# Autodesk Inventor assembly: Car
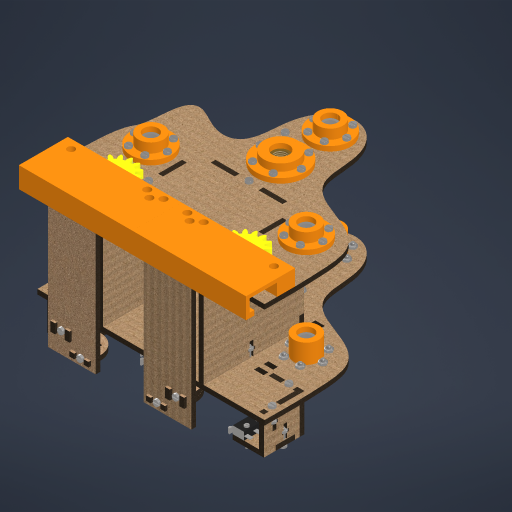
[picture p0: Inventor's stored thumbnail of the model, 512x512]
Saved by Autodesk Inventor 2024.1 (Build 281209000, 209)
## iProperties
Created: 2023-08-04
Part Number: Car
Document SubType Name: Assembly
Designer: jaege
Author: jaege
## Documents named in this file (35)
- C:\Users\jaege\VUB\Schakel_Ind_Elo\Year_1_Both\BA_Thesis\3D_Files\Lift_V2\Car_ASM.iam
- C:\Users\jaege\VUB\Schakel_Ind_Elo\Year_1_Both\BA_Thesis\3D_Files\Lift_V2\Cart_Floor.ipt
- C:\Users\jaege\VUB\Schakel_Ind_Elo\Year_1_Both\BA_Thesis\3D_Files\Lift_V2\Spindle_Block_ASM.iam
- C:\Users\jaege\VUB\Schakel_Ind_Elo\Year_1_Both\BA_Thesis\3D_Files\Lift_V2\Servo_Motor.ipt
- C:\Users\jaege\VUB\Schakel_Ind_Elo\Year_1_Both\BA_Thesis\3D_Files\Lift_V2\Bearing_ASM.iam
- C:\Users\jaege\VUB\Schakel_Ind_Elo\Year_1_Both\BA_Thesis\3D_Files\Lift_V2\Door.ipt
- C:\Users\jaege\VUB\Schakel_Ind_Elo\Year_1_Both\BA_Thesis\3D_Files\Lift_V2\Gear.ipt
- C:\Users\jaege\VUB\Schakel_Ind_Elo\Year_1_Both\BA_Thesis\3D_Files\Lift_V2\Lever.ipt
- C:\Users\jaege\VUB\Schakel_Ind_Elo\Year_1_Both\BA_Thesis\3D_Files\Lift_V2\Receptacle.ipt
- C:\Users\jaege\VUB\Schakel_Ind_Elo\Year_1_Both\BA_Thesis\3D_Files\Lift_V2\Shaft.ipt
- C:\Users\jaege\Documents\Inventor\Content Center Files\R2024\en-US\ISO 1207(2)\ISO 1207 - M3 x 12.ipt
- C:\Users\jaege\Documents\Inventor\Content Center Files\R2024\en-US\ISO 4032(2)\ISO 4032 - M3 - ISO.ipt
- C:\Users\jaege\Documents\Inventor\Content Center Files\R2024\en-US\ISO 7089\ISO 7089 - 3 - 140 HV(1).ipt
- C:\Users\jaege\Documents\Inventor\Content Center Files\R2024\en-US\ISO 1207(2)\ISO 1207 - M3 x 8.ipt
- C:\Users\jaege\VUB\Schakel_Ind_Elo\Year_1_Both\BA_Thesis\3D_Files\Lift_V2\Shaft_MIR.ipt
- C:\Users\jaege\VUB\Schakel_Ind_Elo\Year_1_Both\BA_Thesis\3D_Files\Lift_V2\Receptacle_MIR.ipt
- C:\Users\jaege\VUB\Schakel_Ind_Elo\Year_1_Both\BA_Thesis\3D_Files\Lift_V2\Door_MIR.ipt
- C:\Users\jaege\VUB\Schakel_Ind_Elo\Year_1_Both\BA_Thesis\3D_Files\Lift_V2\Car_Left.ipt
- C:\Users\jaege\VUB\Schakel_Ind_Elo\Year_1_Both\BA_Thesis\3D_Files\Lift_V2\Car_Rear.ipt
- C:\Users\jaege\VUB\Schakel_Ind_Elo\Year_1_Both\BA_Thesis\3D_Files\Lift_V2\Cart_Floor_Bottom.ipt
- C:\Users\jaege\VUB\Schakel_Ind_Elo\Year_1_Both\BA_Thesis\3D_Files\Lift_V2\Spindle_Block_ASM_MIR.iam
- C:\Users\jaege\VUB\Schakel_Ind_Elo\Year_1_Both\BA_Thesis\3D_Files\Lift_V2\Bearing_ASM_MIR1.iam
- C:\Users\jaege\VUB\Schakel_Ind_Elo\Year_1_Both\BA_Thesis\3D_Files\Lift_V2\Magnet_Holder.ipt
- C:\Users\jaege\VUB\Schakel_Ind_Elo\Year_1_Both\BA_Thesis\3D_Files\Lift_V2\LimitSwitch_Small.ipt
- C:\Users\jaege\VUB\Schakel_Ind_Elo\Year_1_Both\BA_Thesis\3D_Files\Lift_V2\Door_LimitSwitch_Offset.ipt
- C:\Users\jaege\VUB\Schakel_Ind_Elo\Year_1_Both\BA_Thesis\3D_Files\Lift_V2\Door_LimitSwitch_Holder_Side_1.ipt
- C:\Users\jaege\VUB\Schakel_Ind_Elo\Year_1_Both\BA_Thesis\3D_Files\Lift_V2\Door_LimitSwitch_Holder_Side_2.ipt
- C:\Users\jaege\VUB\Schakel_Ind_Elo\Year_1_Both\BA_Thesis\3D_Files\Lift_V2\Door_LimitSwitch_Holder_Plate.ipt
- C:\Users\jaege\VUB\Schakel_Ind_Elo\Year_1_Both\BA_Thesis\3D_Files\Lift_V2\Door_LimitSwitch_Holder_Side_1_MIR.ipt
- C:\Users\jaege\VUB\Schakel_Ind_Elo\Year_1_Both\BA_Thesis\3D_Files\Lift_V2\Door_LimitSwitch_Holder_Side_2_MIR.ipt
- C:\Users\jaege\VUB\Schakel_Ind_Elo\Year_1_Both\BA_Thesis\3D_Files\Lift_V2\Door_LimitSwitch_Holder_Plate_MIR.ipt
- C:\Users\jaege\Documents\Inventor\Content Center Files\R2024\en-US\AS 1427(10)\AS 1427 - M2 x 25(7).ipt
- C:\Users\jaege\Documents\Inventor\Content Center Files\R2024\en-US\ISO 7089\ISO 7089 - 2 - 140 HV(1).ipt
- C:\Users\jaege\Documents\Inventor\Content Center Files\R2024\en-US\ISO 4032(2)\ISO 4032 - M2 - ISO.ipt
- C:\Users\jaege\Documents\Inventor\Content Center Files\R2024\en-US\AS 1427(10)\AS 1427 - M2 x 16(7).ipt
## Components (234 placed, 35 different names)
1. Spindle_Block_ASM:1 [sub-assembly]
2. Servo_Motor:1 — Mate:433, Mate:434, Mate:435
3. Bearing_ASM:1 [sub-assembly]
4. Bearing_ASM:2 [sub-assembly]
5. Door:1 — Mate:245, Mate:246, Mate:295, Mate:296, Mate:297, Mate:312, Mate:313, Mate:314, Mate:316, Mate:317, Mate:318
6. Gear:1
7. Lever:1 — Mate:245
8. Lever:2 — Mate:246, Mate:311, Mate:319
9. Receptacle:1 — Angle:20
10. Shaft:1
11. Bearing_ASM:3 [sub-assembly]
12. Servo_Motor:2 — Mate:436, Mate:437
13. Gear:2
14. Shaft_MIR:1
15. Receptacle_MIR:1 — Angle:21, Angle:23, Mate:438, Mate:439, Mate:440, Mate:441, Mate:442, Mate:443, Mate:444, Mate:446, Mate:448, Mate:450, Mate:451, Mate:452, Mate:453, Mate:454
16. Door_MIR:1 — Mate:299, Mate:300, Mate:320, Mate:321, Mate:322, Mate:324, Mate:325, Mate:326
17. Lever:3 — Mate:294, Mate:301, Mate:323
18. Lever:4 — Mate:298
19. Cart_Floor:1 — Flush:6, Mate:166, Mate:167, Mate:168, Mate:169, Flush:8, Symmetry:1, Mate:261, Mate:263, Mate:278, Mate:393, Mate:394, Mate:395, Mate:405, Mate:406, Mate:407, Mate:408, Mate:409, Mate:410, Mate:411, Mate:413, Mate:415, Mate:429, Mate:430, Mate:431, Mate:432, Mate:445, Mate:447, Mate:449, Mate:450, Mate:451, Mate:455
20. Car_Left:1 — Flush:6, Flush:7, Mate:262, Mate:263, Mate:264, Symmetry:2, Mate:412, Mate:414, Mate:416, Angle:13, Angle:15
21. Car_Right:2 — Mate:166, Mate:167, Mate:168, Mate:169, Symmetry:2, Mate:402, Mate:404, Angle:12, Angle:14, Angle:16
22. Car_Rear:1 — Flush:7, Mate:170, Mate:171, Mate:261, Mate:262, Mate:397, Mate:398, Mate:399, Mate:400, Mate:401, Mate:403, Mate:424, Mate:426, Mate:428, Angle:17, Angle:18
23. Cart_Floor_Bottom:1 — Mate:170, Mate:171, Flush:8, Symmetry:1, Mate:244, Flush:9, Mate:247, Mate:264, Mate:265, Mate:266, Mate:267, Mate:268, Mate:269, Mate:270, Mate:271, Mate:272, Mate:273, Mate:274, Mate:275, Mate:276, Mate:277, Mate:279, Mate:280, Mate:281, Mate:282, Mate:283, Mate:284, Flush:35, Mate:285, Mate:286, Mate:287, Flush:36, Mate:288, Mate:305, Mate:307, Mate:331, Mate:335, Mate:339, Mate:343, Mate:360, Mate:361, Mate:362, Mate:364, Mate:365, Mate:366, Mate:376, Mate:377, Mate:378, Mate:380, Mate:381, Mate:382, Mate:383, Mate:417, Mate:418, Mate:419, Mate:420, Mate:421, Mate:422, Mate:423, Mate:425, Mate:427
24. Spindle_Block_ASM_MIR:1 [sub-assembly] — Mate:181, Mate:182, Mate:183, Mate:184, Mate:185, Mate:186, Mate:187, Mate:188, Mate:189, Mate:208, Mate:209, Mate:210, Mate:211, Mate:212, Mate:213, Mate:214, Mate:215, Mate:216, Mate:265, Mate:266
25. Bearing_ASM_MIR1:1 [sub-assembly] — Mate:190, Mate:191, Mate:192, Mate:193, Mate:194, Mate:195, Mate:196, Mate:197, Mate:198, Mate:199, Mate:200, Mate:201, Mate:202, Mate:203, Mate:204, Mate:205, Mate:206, Mate:207, Mate:271, Mate:274
26. Bearing_ASM_MIR1:2 [sub-assembly] — Mate:172, Mate:173, Mate:174, Mate:175, Mate:176, Mate:177, Mate:178, Mate:179, Mate:180, Mate:217, Mate:218, Mate:219, Mate:220, Mate:221, Mate:222, Mate:223, Mate:224, Mate:225, Mate:267, Mate:268
27. Bearing_ASM_MIR1:3 [sub-assembly] — Mate:226, Mate:227, Mate:228, Mate:229, Mate:230, Mate:231, Mate:232, Mate:233, Mate:234, Mate:235, Mate:236, Mate:237, Mate:238, Mate:239, Mate:240, Mate:241, Mate:242, Mate:243, Mate:272, Mate:273
28. LimitSwitch_Small:1 — Mate:250, Mate:251, Mate:252, Mate:258, Mate:259, Mate:260
29. LimitSwitch_Small:6 — Mate:308, Mate:309, Mate:310, Mate:311, Mate:344, Mate:345, Mate:346, Mate:348, Mate:349, Mate:350
30. LimitSwitch_Small:3 — Mate:258, Mate:259, Mate:260, Mate:281, Mate:282, Mate:328, Mate:329, Mate:330, Mate:332, Mate:333, Mate:334
31. LimitSwitch_Small:4 — Mate:255, Mate:256, Mate:257, Mate:283, Mate:284, Mate:336, Mate:337, Mate:338, Mate:340, Mate:341, Mate:342
32. LimitSwitch_Small:5 — Mate:290, Mate:291, Mate:292, Mate:294, Mate:301, Mate:352, Mate:353, Mate:354, Mate:356, Mate:357, Mate:358
33. LimitSwitch_Small:2 — Mate:249, Mate:253, Mate:254, Mate:255, Mate:256, Mate:257
34. Magnet_Holder:1 — Mate:244, Mate:278, Mate:279, Mate:280, Mate:396, Angle:19
35. Door_LimitSwitch_Offset:1 — Flush:9, Mate:248, Flush:10, Mate:249, Mate:253, Mate:254
36. Door_LimitSwitch_Offset:2 — Mate:247, Mate:248, Flush:10, Mate:250, Mate:251, Mate:252
37. Door_LimitSwitch_Holder_Side_1:1 — Flush:35, Mate:285, Mate:286, Mate:287, Mate:289, Flush:37, Flush:38, Flush:39, Mate:367, Mate:371, Angle:10
38. Door_LimitSwitch_Holder_Side_2:1 — Flush:36, Mate:288, Mate:289, Flush:37, Mate:293, Flush:40, Mate:363, Mate:375, Angle:8
39. Door_LimitSwitch_Holder_Plate:1 — Flush:38, Mate:290, Mate:291, Mate:292, Mate:293, Flush:39, Flush:40, Mate:355, Mate:359, Mate:368, Mate:369, Mate:370, Mate:372, Mate:373, Mate:374
40. Lever:5 — Mate:295, Mate:296, Mate:297, Mate:315, Angle:6
41. Lever:6 — Mate:298, Mate:299, Mate:300, Mate:327
42. Door_LimitSwitch_Holder_Side_1_MIR:1 — Flush:41, Mate:302, Flush:43, Mate:304, Mate:305, Flush:44, Mate:307, Mate:380, Mate:384, Mate:388, Angle:2
43. Door_LimitSwitch_Holder_Side_2_MIR:1 — Flush:41, Mate:302, Flush:42, Mate:303, Flush:44, Mate:379, Mate:392, Angle:3
44. Door_LimitSwitch_Holder_Plate_MIR:1 — Flush:42, Flush:43, Mate:303, Mate:304, Mate:308, Mate:309, Mate:310, Mate:347, Mate:351, Mate:385, Mate:386, Mate:387, Mate:389, Mate:390, Mate:391
45. ISO 1207 M3 x 12:53 — Mate:312, Mate:313
46. ISO 4032 M3:53 — Mate:314, Mate:315, Angle:5, Angle:6, Angle:11
47. ISO 1207 M3 x 12:54 — Mate:316, Mate:317
48. ISO 4032 M3:54 — Mate:318, Mate:319, Angle:5, Angle:11
49. ISO 1207 M3 x 12:55 — Mate:320, Mate:321
50. ISO 4032 M3:55 — Mate:322, Mate:323
51. ISO 1207 M3 x 12:56 — Mate:324, Mate:325
52. ISO 4032 M3:56 — Mate:326, Mate:327
53. AS 1427 (8) - Metric M2 x 25:1 — Mate:328, Mate:329
54. ISO 7089 2:1 — Mate:330, Mate:331, Insert:5
55. ISO 4032 M2:1 — Insert:5
56. AS 1427 (8) - Metric M2 x 25:2 — Mate:332, Mate:333
57. ISO 7089 2:2 — Mate:334, Mate:335, Insert:6
58. ISO 4032 M2:2 — Insert:6
59. AS 1427 (8) - Metric M2 x 25:3 — Mate:336, Mate:337
60. ISO 7089 2:3 — Mate:338, Mate:339, Insert:7
61. ISO 4032 M2:3 — Insert:7
62. AS 1427 (8) - Metric M2 x 25:4 — Mate:340, Mate:341
63. ISO 7089 2:4 — Mate:342, Mate:343, Insert:8
64. ISO 4032 M2:4 — Insert:8
65. AS 1427 (8) - Metric M2 x 16:1 — Mate:344, Mate:345
66. ISO 7089 2:5 — Mate:346, Mate:347, Insert:9
67. ISO 4032 M2:5 — Insert:9
68. AS 1427 (8) - Metric M2 x 16:2 — Mate:348, Mate:349
69. ISO 7089 2:6 — Mate:350, Mate:351, Insert:10
70. ISO 4032 M2:6 — Insert:10
71. AS 1427 (8) - Metric M2 x 16:3 — Mate:352, Mate:353
72. ISO 7089 2:7 — Mate:354, Mate:355, Insert:11
73. ISO 4032 M2:7 — Insert:11
74. AS 1427 (8) - Metric M2 x 16:4 — Mate:356, Mate:357
75. ISO 7089 2:8 — Mate:358, Mate:359, Insert:12
76. ISO 4032 M2:8 — Insert:12
77. ISO 1207 M3 x 12:57 — Mate:360, Mate:361
78. ISO 4032 M3:57 — Mate:362, Mate:363, Angle:7, Angle:8
79. ISO 1207 M3 x 12:58 — Mate:364, Mate:365
80. ISO 4032 M3:58 — Mate:366, Mate:367, Angle:9, Angle:10
81. ISO 1207 M3 x 12:59 — Mate:368, Mate:369
82. ISO 4032 M3:59 — Mate:370, Mate:371, Angle:9
83. ISO 1207 M3 x 12:60 — Mate:372, Mate:373
84. ISO 4032 M3:60 — Mate:374, Mate:375, Angle:7
85. ISO 1207 M3 x 12:61 — Mate:376, Mate:377
86. ISO 4032 M3:61 — Mate:378, Mate:379, Angle:4
87. ISO 1207 M3 x 12:62 — Mate:381, Mate:382
88. ISO 4032 M3:62 — Mate:383, Mate:384, Angle:1
89. ISO 1207 M3 x 12:63 — Mate:385, Mate:386
90. ISO 4032 M3:63 — Mate:387, Mate:388, Angle:1, Angle:2
91. ISO 1207 M3 x 12:64 — Mate:389, Mate:390
92. ISO 4032 M3:64 — Mate:391, Mate:392, Angle:3, Angle:4
93. ISO 1207 M3 x 12:65 — Mate:393, Mate:394
94. ISO 4032 M3:65 — Mate:395, Mate:396, Angle:19
95. ISO 1207 M3 x 12:66 — Mate:397, Mate:398
96. ISO 4032 M3:66 — Mate:401, Mate:402, Angle:16
97. ISO 1207 M3 x 12:67 — Mate:399, Mate:400
98. ISO 4032 M3:67 — Mate:403, Mate:404
99. ISO 1207 M3 x 12:68 — Mate:405, Mate:406
100. ISO 4032 M3:68 — Mate:411, Mate:412, Angle:15
101. ISO 1207 M3 x 12:69 — Mate:407, Mate:408, Angle:26
102. ISO 1207 M3 x 12:70 — Mate:409, Mate:410
103. ISO 4032 M3:69 — Mate:413, Mate:414, Angle:17
104. ISO 4032 M3:70 — Mate:415, Mate:416, Angle:14
105. ISO 1207 M3 x 12:71 — Mate:417, Mate:418
106. ISO 4032 M3:71 — Mate:423, Mate:424, Angle:18
107. ISO 1207 M3 x 12:72 — Mate:419, Mate:420
108. ISO 1207 M3 x 12:73 — Mate:421, Mate:422
109. ISO 4032 M3:72 — Mate:425, Mate:426, Angle:13
110. ISO 4032 M3:73 — Mate:427, Mate:428, Angle:12
111. ISO 1207 M3 x 8:3 — Mate:429, Mate:430, Mate:437
112. ISO 1207 M3 x 8:4 — Mate:431, Mate:432, Mate:436
113. ISO 1207 M3 x 12:74 — Mate:438, Mate:439
114. ISO 7089 3:5 — Mate:444, Mate:445, Insert:13
115. ISO 4032 M3:74 — Insert:13
116. ISO 1207 M3 x 12:75 — Mate:440, Mate:441
117. ISO 1207 M3 x 12:76 — Mate:442, Mate:443
118. ISO 7089 3:6 — Mate:446, Mate:447, Insert:14
119. ISO 7089 3:7 — Mate:448, Mate:449, Insert:15
120. ISO 4032 M3:75 — Insert:14
121. ISO 4032 M3:76 — Insert:15
122. ISO 1207 M3 x 12:77 — Mate:452, Mate:453
123. ISO 7089 3:8 — Mate:454, Mate:455, Insert:16
124. ISO 4032 M3:77 — Insert:16
125. ISO 1207 M3 x 12:29 — Mate:226, Mate:227
126. ISO 4032 M3:29 — Mate:228, Flush:14
127. ISO 1207 M3 x 12:30 — Mate:229, Mate:230
128. ISO 4032 M3:30 — Mate:231, Flush:15, Angle:24
129. ISO 1207 M3 x 12:31 — Mate:232, Mate:233, Mate:276
130. ISO 4032 M3:31 — Mate:234, Flush:11, Flush:14, Flush:16, Flush:17
131. ISO 1207 M3 x 12:32 — Mate:235, Mate:236
132. ISO 4032 M3:32 — Mate:237, Flush:13, Angle:23, Angle:24, Angle:25
133. ISO 1207 M3 x 12:33 — Mate:238, Mate:239
134. ISO 4032 M3:33 — Mate:240, Mate:277, Flush:11, Flush:12, Flush:15, Flush:16
135. ISO 1207 M3 x 12:34 — Mate:241, Mate:242
136. ISO 4032 M3:34 — Mate:243, Flush:12, Flush:13, Angle:25
137. ISO 1207 M3 x 12:35 — Mate:172, Mate:173
138. ISO 4032 M3:35 — Mate:174, Flush:18, Flush:21
139. ISO 1207 M3 x 12:36 — Mate:175, Mate:176, Mate:269
140. ISO 4032 M3:36 — Mate:177, Flush:17, Flush:18, Flush:19
141. ISO 1207 M3 x 12:37 — Mate:178, Mate:179
142. ISO 4032 M3:37 — Mate:180, Flush:21, Flush:22
143. ISO 1207 M3 x 12:38 — Mate:181, Mate:182, Mate:270
144. ISO 4032 M3:38 — Mate:183, Flush:26
145. ISO 1207 M3 x 12:39 — Mate:184, Mate:185
146. ISO 4032 M3:39 — Mate:186, Flush:24, Flush:27
147. ISO 1207 M3 x 12:40 — Mate:187, Mate:188
148. ISO 4032 M3:40 — Mate:189, Flush:27, Flush:28, Flush:34
149. ISO 4032 M3:41 — Mate:192, Flush:31, Flush:32
150. ISO 1207 M3 x 12:41 — Mate:190, Mate:191
151. ISO 1207 M3 x 12:42 — Mate:193, Mate:194, Mate:275
152. ISO 4032 M3:42 — Mate:195, Flush:30, Flush:31
153. ISO 1207 M3 x 12:43 — Mate:196, Mate:197
154. ISO 4032 M3:43 — Mate:198, Flush:32, Flush:33
155. ISO 1207 M3 x 12:44 — Mate:199, Mate:200
156. ISO 4032 M3:44 — Mate:201, Flush:29, Flush:30, Flush:34
157. ISO 1207 M3 x 12:45 — Mate:202, Mate:203
158. ISO 4032 M3:45 — Mate:204, Flush:29
159. ISO 1207 M3 x 12:46 — Mate:205, Mate:206
160. ISO 4032 M3:46 — Mate:207, Flush:33
161. ISO 1207 M3 x 12:47 — Mate:208, Mate:209
162. ISO 4032 M3:47 — Mate:210, Flush:22, Flush:23
163. ISO 1207 M3 x 12:48 — Mate:211, Mate:212
164. ISO 4032 M3:48 — Mate:213, Flush:23
165. ISO 1207 M3 x 12:49 — Mate:214, Mate:215
166. ISO 4032 M3:49 — Mate:216, Flush:28
167. ISO 1207 M3 x 12:50 — Mate:217, Mate:218
168. ISO 4032 M3:50 — Mate:219, Flush:19, Flush:20
169. ISO 1207 M3 x 12:51 — Mate:220, Mate:221
170. ISO 4032 M3:51 — Mate:222, Flush:20, Flush:24, Flush:25
171. ISO 1207 M3 x 12:52 — Mate:223, Mate:224
172. ISO 4032 M3:52 — Mate:225, Flush:25, Flush:26
173. ISO 1207 M3 x 12:23
174. ISO 4032 M3:23
175. ISO 1207 M3 x 12:24
176. ISO 4032 M3:24
177. ISO 1207 M3 x 12:25
178. ISO 4032 M3:25
179. ISO 1207 M3 x 12:26
180. ISO 4032 M3:26
181. ISO 1207 M3 x 12:27
182. ISO 4032 M3:27
183. ISO 1207 M3 x 12:28
184. ISO 4032 M3:28
185. ISO 1207 M3 x 12:1
186. ISO 4032 M3:1
187. ISO 1207 M3 x 12:2
188. ISO 4032 M3:2
189. ISO 1207 M3 x 12:3
190. ISO 4032 M3:3
191. ISO 1207 M3 x 12:4
192. ISO 4032 M3:4
193. ISO 1207 M3 x 12:5
194. ISO 4032 M3:5
195. ISO 1207 M3 x 12:6 — Angle:20, Angle:26
196. ISO 4032 M3:6
197. ISO 4032 M3:7
198. ISO 1207 M3 x 12:7
199. ISO 1207 M3 x 12:8
200. ISO 7089 3:1
201. ISO 4032 M3:8
202. ISO 1207 M3 x 12:9
203. ISO 7089 3:2
204. ISO 4032 M3:9
205. ISO 1207 M3 x 12:10
206. ISO 7089 3:3
207. ISO 4032 M3:10
208. ISO 1207 M3 x 12:11
209. ISO 7089 3:4
210. ISO 4032 M3:11
211. ISO 1207 M3 x 8:1 — Mate:433, Mate:435
212. ISO 1207 M3 x 8:2 — Mate:434
213. ISO 1207 M3 x 12:12
214. ISO 4032 M3:12
215. ISO 1207 M3 x 12:13
216. ISO 4032 M3:13
217. ISO 1207 M3 x 12:14
218. ISO 4032 M3:14
219. ISO 1207 M3 x 12:15
220. ISO 4032 M3:15
221. ISO 1207 M3 x 12:16
222. ISO 4032 M3:16
223. ISO 1207 M3 x 12:17
224. ISO 4032 M3:17
225. ISO 1207 M3 x 12:18 — Angle:22
226. ISO 4032 M3:18
227. ISO 1207 M3 x 12:19 — Angle:21, Angle:22
228. ISO 4032 M3:19
229. ISO 1207 M3 x 12:20
230. ISO 4032 M3:20
231. ISO 1207 M3 x 12:21
232. ISO 4032 M3:21
233. ISO 1207 M3 x 12:22
234. ISO 4032 M3:22
## Relationships (533: Mate 445, Flush 44, Angle 26, Insert 16, Symmetry 2)
- [Mate] (0.25 mm): Receptacle:1 ↔ Shaft:1
- [Mate] (0.25 mm): Receptacle:1 ↔ Shaft:1
- [Mate]: Servo_Motor:1 ↔ Cart_Floor:1
- [Mate]: Bearing_ASM:1 ↔ Cart_Floor:1
- [Mate]: Bearing_ASM:1 ↔ Cart_Floor:1
- [Mate]: Bearing_ASM:1 ↔ Cart_Floor:1
- [Mate]: Bearing_ASM:2 ↔ Cart_Floor:1
- [Mate]: Bearing_ASM:2 ↔ Cart_Floor:1
- [Mate]: Bearing_ASM:2 ↔ Cart_Floor:1
- [Mate]: Spindle_Block_ASM:1 ↔ Cart_Floor:1
- [Mate]: Spindle_Block_ASM:1 ↔ Cart_Floor:1
- [Mate]: Spindle_Block_ASM:1 ↔ Cart_Floor:1
- [Mate]: Servo_Motor:1 ↔ Gear:1
- [Mate]: Servo_Motor:1 ↔ Gear:1
- [Mate]: Receptacle:1 ↔ Cart_Floor:1
- [Flush]: Receptacle:1 ↔ Cart_Floor:1
- [Flush]: Receptacle:1 ↔ Shaft:1
- [Flush]: Receptacle:1 ↔ Shaft:1
- [Mate] (0.25 mm): Shaft:1 ↔ Cart_Floor:1
- [Mate]: Bearing_ASM:2 ↔ ISO 1207 M3 x 12:1
- [Mate]: Bearing_ASM:2 ↔ ISO 1207 M3 x 12:1
- [Mate]: Bearing_ASM:2 ↔ ISO 4032 M3:1
- [Mate]: Cart_Floor:1 ↔ ISO 4032 M3:1
- [Mate]: Bearing_ASM:2 ↔ ISO 1207 M3 x 12:2
- [Mate]: Bearing_ASM:2 ↔ ISO 1207 M3 x 12:2
- [Mate]: Bearing_ASM:2 ↔ ISO 4032 M3:2
- [Mate]: Cart_Floor:1 ↔ ISO 4032 M3:2
- [Mate]: Bearing_ASM:2 ↔ ISO 1207 M3 x 12:3
- [Mate]: Bearing_ASM:2 ↔ ISO 1207 M3 x 12:3
- [Mate]: Bearing_ASM:2 ↔ ISO 4032 M3:3
- [Mate]: Cart_Floor:1 ↔ ISO 4032 M3:3
- [Mate]: Spindle_Block_ASM:1 ↔ ISO 1207 M3 x 12:4
- [Mate]: Spindle_Block_ASM:1 ↔ ISO 1207 M3 x 12:4
- [Mate]: Spindle_Block_ASM:1 ↔ ISO 4032 M3:4
- [Mate]: Cart_Floor:1 ↔ ISO 4032 M3:4
- [Mate]: Spindle_Block_ASM:1 ↔ ISO 1207 M3 x 12:5
- [Mate]: Spindle_Block_ASM:1 ↔ ISO 1207 M3 x 12:5
- [Mate]: Spindle_Block_ASM:1 ↔ ISO 4032 M3:5
- [Mate]: Cart_Floor:1 ↔ ISO 4032 M3:5
- [Mate]: Spindle_Block_ASM:1 ↔ ISO 1207 M3 x 12:6
- [Mate]: Spindle_Block_ASM:1 ↔ ISO 1207 M3 x 12:6
- [Mate]: Spindle_Block_ASM:1 ↔ ISO 4032 M3:6
- [Mate]: Cart_Floor:1 ↔ ISO 4032 M3:6
- [Mate]: Bearing_ASM:1 ↔ ISO 1207 M3 x 12:7
- [Mate]: Bearing_ASM:1 ↔ ISO 1207 M3 x 12:7
- [Mate]: Bearing_ASM:1 ↔ ISO 4032 M3:7
- [Mate]: Cart_Floor:1 ↔ ISO 4032 M3:7
- [Mate]: Receptacle:1 ↔ ISO 1207 M3 x 12:8
- [Mate]: Receptacle:1 ↔ ISO 1207 M3 x 12:8
- [Mate]: Receptacle:1 ↔ ISO 7089 3:1
- [Mate]: Cart_Floor:1 ↔ ISO 7089 3:1
- [Insert]: ISO 7089 3:1 ↔ ISO 4032 M3:8
- [Mate]: Receptacle:1 ↔ ISO 1207 M3 x 12:9
- [Mate]: Receptacle:1 ↔ ISO 1207 M3 x 12:9
- [Mate]: Receptacle:1 ↔ ISO 7089 3:2
- [Mate]: Cart_Floor:1 ↔ ISO 7089 3:2
- [Insert]: ISO 7089 3:2 ↔ ISO 4032 M3:9
- [Mate]: Receptacle:1 ↔ ISO 1207 M3 x 12:10
- [Mate]: Receptacle:1 ↔ ISO 1207 M3 x 12:10
- [Mate]: Receptacle:1 ↔ ISO 7089 3:3
- [Mate]: Cart_Floor:1 ↔ ISO 7089 3:3
- [Insert]: ISO 7089 3:3 ↔ ISO 4032 M3:10
- [Mate]: Receptacle:1 ↔ ISO 1207 M3 x 12:11
- [Mate]: Receptacle:1 ↔ ISO 1207 M3 x 12:11
- [Mate]: Receptacle:1 ↔ ISO 7089 3:4
- [Mate]: Cart_Floor:1 ↔ ISO 7089 3:4
- [Insert]: ISO 7089 3:4 ↔ ISO 4032 M3:11
- [Mate]: Cart_Floor:1 ↔ ISO 1207 M3 x 8:1
- [Mate]: Cart_Floor:1 ↔ ISO 1207 M3 x 8:1
- [Mate]: Cart_Floor:1 ↔ ISO 1207 M3 x 8:2
- [Mate]: Cart_Floor:1 ↔ ISO 1207 M3 x 8:2
- [Mate]: Door:1 ↔ Lever:2
- [Mate]: Door:1 ↔ Lever:2
- [Mate]: Door:1 ↔ Lever:1
- [Mate]: Door:1 ↔ Lever:1
- [Mate]: Bearing_ASM:1 ↔ ISO 1207 M3 x 12:12
- [Mate]: Bearing_ASM:1 ↔ ISO 1207 M3 x 12:12
- [Mate]: Bearing_ASM:1 ↔ ISO 4032 M3:12
- [Mate]: Cart_Floor:1 ↔ ISO 4032 M3:12
- [Mate]: Bearing_ASM:1 ↔ ISO 1207 M3 x 12:13
- [Mate]: Bearing_ASM:1 ↔ ISO 1207 M3 x 12:13
- [Mate]: Bearing_ASM:1 ↔ ISO 4032 M3:13
- [Mate]: Cart_Floor:1 ↔ ISO 4032 M3:13
- [Mate]: Bearing_ASM:1 ↔ ISO 1207 M3 x 12:14
- [Mate]: Bearing_ASM:1 ↔ ISO 1207 M3 x 12:14
- [Mate]: Bearing_ASM:1 ↔ ISO 4032 M3:14
- [Mate]: Cart_Floor:1 ↔ ISO 4032 M3:14
- [Mate]: Bearing_ASM:1 ↔ ISO 1207 M3 x 12:15
- [Mate]: Bearing_ASM:1 ↔ ISO 1207 M3 x 12:15
- [Mate]: Bearing_ASM:1 ↔ ISO 4032 M3:15
- [Mate]: Cart_Floor:1 ↔ ISO 4032 M3:15
- [Mate]: Bearing_ASM:1 ↔ ISO 1207 M3 x 12:16
- [Mate]: Bearing_ASM:1 ↔ ISO 1207 M3 x 12:16
- [Mate]: Bearing_ASM:1 ↔ ISO 4032 M3:16
- [Mate]: Cart_Floor:1 ↔ ISO 4032 M3:16
- [Mate]: Spindle_Block_ASM:1 ↔ ISO 1207 M3 x 12:17
- [Mate]: Spindle_Block_ASM:1 ↔ ISO 1207 M3 x 12:17
- [Mate]: Spindle_Block_ASM:1 ↔ ISO 4032 M3:17
- [Mate]: Cart_Floor:1 ↔ ISO 4032 M3:17
- [Mate]: Spindle_Block_ASM:1 ↔ ISO 1207 M3 x 12:18
- [Mate]: Spindle_Block_ASM:1 ↔ ISO 1207 M3 x 12:18
- [Mate]: Spindle_Block_ASM:1 ↔ ISO 4032 M3:18
- [Mate]: Cart_Floor:1 ↔ ISO 4032 M3:18
- [Mate]: Spindle_Block_ASM:1 ↔ ISO 1207 M3 x 12:19
- [Mate]: Spindle_Block_ASM:1 ↔ ISO 1207 M3 x 12:19
- [Mate]: Spindle_Block_ASM:1 ↔ ISO 4032 M3:19
- [Mate]: Cart_Floor:1 ↔ ISO 4032 M3:19
- [Mate]: Bearing_ASM:2 ↔ ISO 1207 M3 x 12:20
- [Mate]: Bearing_ASM:2 ↔ ISO 1207 M3 x 12:20
- [Mate]: Bearing_ASM:2 ↔ ISO 4032 M3:20
- [Mate]: Cart_Floor:1 ↔ ISO 4032 M3:20
- [Mate]: Bearing_ASM:2 ↔ ISO 1207 M3 x 12:21
- [Mate]: Bearing_ASM:2 ↔ ISO 1207 M3 x 12:21
- [Mate]: Bearing_ASM:2 ↔ ISO 4032 M3:21
- [Mate]: Cart_Floor:1 ↔ ISO 4032 M3:21
- [Mate]: Bearing_ASM:2 ↔ ISO 1207 M3 x 12:22
- [Mate]: Bearing_ASM:2 ↔ ISO 1207 M3 x 12:22
- [Mate]: Bearing_ASM:2 ↔ ISO 4032 M3:22
- [Mate]: Cart_Floor:1 ↔ ISO 4032 M3:22
- [Mate]: Bearing_ASM:3 ↔ Cart_Floor:1
- [Mate]: Bearing_ASM:3 ↔ Cart_Floor:1
- [Mate]: Bearing_ASM:3 ↔ Cart_Floor:1
- [Mate]: Bearing_ASM:3 ↔ ISO 1207 M3 x 12:23
- [Mate]: Bearing_ASM:3 ↔ ISO 1207 M3 x 12:23
- [Mate]: Bearing_ASM:3 ↔ ISO 4032 M3:23
- [Mate]: Cart_Floor:1 ↔ ISO 4032 M3:23
- [Mate]: Bearing_ASM:3 ↔ ISO 1207 M3 x 12:24
- [Mate]: Bearing_ASM:3 ↔ ISO 1207 M3 x 12:24
- [Mate]: Bearing_ASM:3 ↔ ISO 4032 M3:24
- [Mate]: Cart_Floor:1 ↔ ISO 4032 M3:24
- [Mate]: Bearing_ASM:3 ↔ ISO 1207 M3 x 12:25
- [Mate]: Bearing_ASM:3 ↔ ISO 1207 M3 x 12:25
- [Mate]: Bearing_ASM:3 ↔ ISO 4032 M3:25
- [Mate]: Cart_Floor:1 ↔ ISO 4032 M3:25
- [Mate]: Bearing_ASM:3 ↔ ISO 1207 M3 x 12:26
- [Mate]: Bearing_ASM:3 ↔ ISO 1207 M3 x 12:26
- [Mate]: Bearing_ASM:3 ↔ ISO 4032 M3:26
- [Mate]: Cart_Floor:1 ↔ ISO 4032 M3:26
- [Mate]: Bearing_ASM:3 ↔ ISO 1207 M3 x 12:27
- [Mate]: Bearing_ASM:3 ↔ ISO 1207 M3 x 12:27
- [Mate]: Bearing_ASM:3 ↔ ISO 4032 M3:27
- [Mate]: Cart_Floor:1 ↔ ISO 4032 M3:27
- [Mate]: Bearing_ASM:3 ↔ ISO 1207 M3 x 12:28
- [Mate]: Bearing_ASM:3 ↔ ISO 1207 M3 x 12:28
- [Mate]: Bearing_ASM:3 ↔ ISO 4032 M3:28
- [Mate]: Cart_Floor:1 ↔ ISO 4032 M3:28
- [Mate]: Servo_Motor:2 ↔ Cart_Floor:1
- [Mate]: Servo_Motor:2 ↔ Gear:2
- [Mate]: Servo_Motor:2 ↔ Gear:2
- [Mate] (0.25 mm): Shaft_MIR:1 ↔ Receptacle_MIR:1
- [Flush]: Shaft_MIR:1 ↔ Receptacle_MIR:1
- [Flush]: Shaft_MIR:1 ↔ Receptacle_MIR:1
- [Mate] (0.25 mm): Shaft_MIR:1 ↔ Receptacle_MIR:1
- [Mate]: Door_MIR:1 ↔ Lever:3
- [Mate]: Door_MIR:1 ↔ Lever:3
- [Mate]: Door_MIR:1 ↔ Lever:4
- [Mate]: Door_MIR:1 ↔ Lever:4
- [Mate]: Door_MIR:1 ↔ Lever:4
- [Mate]: Door_MIR:1 ↔ Lever:3
- [Mate]: Door:1 ↔ Shaft_MIR:1
- [Mate]: Door:1 ↔ Shaft_MIR:1
- [Mate]: Door:1 ↔ Shaft_MIR:1
- [Mate]: Shaft:1 ↔ Door_MIR:1
- [Mate]: Shaft:1 ↔ Door_MIR:1
- [Mate]: Shaft:1 ↔ Door_MIR:1
- Flush:6: Cart_Floor:1 ↔ Car_Left:1
- Mate:166: Cart_Floor:1 ↔ Car_Right:2
- Mate:167: Cart_Floor:1 ↔ Car_Right:2
- Mate:168: Cart_Floor:1 ↔ Car_Right:2
- Mate:169: Cart_Floor:1 ↔ Car_Right:2
- Flush:7: Car_Left:1 ↔ Car_Rear:1
- Mate:170: Car_Rear:1 ↔ Cart_Floor_Bottom:1
- Mate:171: Car_Rear:1 ↔ Cart_Floor_Bottom:1
- Flush:8: Cart_Floor:1 ↔ Cart_Floor_Bottom:1
- Symmetry:1: Cart_Floor:1 ↔ Cart_Floor_Bottom:1
- Mate:172: Bearing_ASM_MIR1:2 ↔ ISO 1207 M3 x 12:35
- Mate:173: Bearing_ASM_MIR1:2 ↔ ISO 1207 M3 x 12:35
- Mate:174: Bearing_ASM_MIR1:2 ↔ ISO 4032 M3:35
- Mate:175: Bearing_ASM_MIR1:2 ↔ ISO 1207 M3 x 12:36
- Mate:176: Bearing_ASM_MIR1:2 ↔ ISO 1207 M3 x 12:36
- Mate:177: Bearing_ASM_MIR1:2 ↔ ISO 4032 M3:36
- Mate:178: Bearing_ASM_MIR1:2 ↔ ISO 1207 M3 x 12:37
- Mate:179: Bearing_ASM_MIR1:2 ↔ ISO 1207 M3 x 12:37
- Mate:180: Bearing_ASM_MIR1:2 ↔ ISO 4032 M3:37
- Mate:181: Spindle_Block_ASM_MIR:1 ↔ ISO 1207 M3 x 12:38
- Mate:182: Spindle_Block_ASM_MIR:1 ↔ ISO 1207 M3 x 12:38
- Mate:183: Spindle_Block_ASM_MIR:1 ↔ ISO 4032 M3:38
- Mate:184: Spindle_Block_ASM_MIR:1 ↔ ISO 1207 M3 x 12:39
- Mate:185: Spindle_Block_ASM_MIR:1 ↔ ISO 1207 M3 x 12:39
- Mate:186: Spindle_Block_ASM_MIR:1 ↔ ISO 4032 M3:39
- Mate:187: Spindle_Block_ASM_MIR:1 ↔ ISO 1207 M3 x 12:40
- Mate:188: Spindle_Block_ASM_MIR:1 ↔ ISO 1207 M3 x 12:40
- Mate:189: Spindle_Block_ASM_MIR:1 ↔ ISO 4032 M3:40
- Mate:190: Bearing_ASM_MIR1:1 ↔ ISO 1207 M3 x 12:41
- Mate:191: Bearing_ASM_MIR1:1 ↔ ISO 1207 M3 x 12:41
- Mate:192: Bearing_ASM_MIR1:1 ↔ ISO 4032 M3:41
- Mate:193: Bearing_ASM_MIR1:1 ↔ ISO 1207 M3 x 12:42
- Mate:194: Bearing_ASM_MIR1:1 ↔ ISO 1207 M3 x 12:42
- Mate:195: Bearing_ASM_MIR1:1 ↔ ISO 4032 M3:42
- Mate:196: Bearing_ASM_MIR1:1 ↔ ISO 1207 M3 x 12:43
- Mate:197: Bearing_ASM_MIR1:1 ↔ ISO 1207 M3 x 12:43
- Mate:198: Bearing_ASM_MIR1:1 ↔ ISO 4032 M3:43
- Mate:199: Bearing_ASM_MIR1:1 ↔ ISO 1207 M3 x 12:44
- Mate:200: Bearing_ASM_MIR1:1 ↔ ISO 1207 M3 x 12:44
- Mate:201: Bearing_ASM_MIR1:1 ↔ ISO 4032 M3:44
- Mate:202: Bearing_ASM_MIR1:1 ↔ ISO 1207 M3 x 12:45
- Mate:203: Bearing_ASM_MIR1:1 ↔ ISO 1207 M3 x 12:45
- Mate:204: Bearing_ASM_MIR1:1 ↔ ISO 4032 M3:45
- Mate:205: Bearing_ASM_MIR1:1 ↔ ISO 1207 M3 x 12:46
- Mate:206: Bearing_ASM_MIR1:1 ↔ ISO 1207 M3 x 12:46
- Mate:207: Bearing_ASM_MIR1:1 ↔ ISO 4032 M3:46
- Mate:208: Spindle_Block_ASM_MIR:1 ↔ ISO 1207 M3 x 12:47
- Mate:209: Spindle_Block_ASM_MIR:1 ↔ ISO 1207 M3 x 12:47
- Mate:210: Spindle_Block_ASM_MIR:1 ↔ ISO 4032 M3:47
- Mate:211: Spindle_Block_ASM_MIR:1 ↔ ISO 1207 M3 x 12:48
- Mate:212: Spindle_Block_ASM_MIR:1 ↔ ISO 1207 M3 x 12:48
- Mate:213: Spindle_Block_ASM_MIR:1 ↔ ISO 4032 M3:48
- Mate:214: Spindle_Block_ASM_MIR:1 ↔ ISO 1207 M3 x 12:49
- Mate:215: Spindle_Block_ASM_MIR:1 ↔ ISO 1207 M3 x 12:49
- Mate:216: Spindle_Block_ASM_MIR:1 ↔ ISO 4032 M3:49
- Mate:217: Bearing_ASM_MIR1:2 ↔ ISO 1207 M3 x 12:50
- Mate:218: Bearing_ASM_MIR1:2 ↔ ISO 1207 M3 x 12:50
- Mate:219: Bearing_ASM_MIR1:2 ↔ ISO 4032 M3:50
- Mate:220: Bearing_ASM_MIR1:2 ↔ ISO 1207 M3 x 12:51
- Mate:221: Bearing_ASM_MIR1:2 ↔ ISO 1207 M3 x 12:51
- Mate:222: Bearing_ASM_MIR1:2 ↔ ISO 4032 M3:51
- Mate:223: Bearing_ASM_MIR1:2 ↔ ISO 1207 M3 x 12:52
- Mate:224: Bearing_ASM_MIR1:2 ↔ ISO 1207 M3 x 12:52
- Mate:225: Bearing_ASM_MIR1:2 ↔ ISO 4032 M3:52
- Mate:226: Bearing_ASM_MIR1:3 ↔ ISO 1207 M3 x 12:29
- Mate:227: Bearing_ASM_MIR1:3 ↔ ISO 1207 M3 x 12:29
- Mate:228: Bearing_ASM_MIR1:3 ↔ ISO 4032 M3:29
- Mate:229: Bearing_ASM_MIR1:3 ↔ ISO 1207 M3 x 12:30
- Mate:230: Bearing_ASM_MIR1:3 ↔ ISO 1207 M3 x 12:30
- Mate:231: Bearing_ASM_MIR1:3 ↔ ISO 4032 M3:30
- Mate:232: Bearing_ASM_MIR1:3 ↔ ISO 1207 M3 x 12:31
- Mate:233: Bearing_ASM_MIR1:3 ↔ ISO 1207 M3 x 12:31
- Mate:234: Bearing_ASM_MIR1:3 ↔ ISO 4032 M3:31
- Mate:235: Bearing_ASM_MIR1:3 ↔ ISO 1207 M3 x 12:32
- Mate:236: Bearing_ASM_MIR1:3 ↔ ISO 1207 M3 x 12:32
- Mate:237: Bearing_ASM_MIR1:3 ↔ ISO 4032 M3:32
- Mate:238: Bearing_ASM_MIR1:3 ↔ ISO 1207 M3 x 12:33
- Mate:239: Bearing_ASM_MIR1:3 ↔ ISO 1207 M3 x 12:33
- Mate:240: Bearing_ASM_MIR1:3 ↔ ISO 4032 M3:33
- Mate:241: Bearing_ASM_MIR1:3 ↔ ISO 1207 M3 x 12:34
- Mate:242: Bearing_ASM_MIR1:3 ↔ ISO 1207 M3 x 12:34
- Mate:243: Bearing_ASM_MIR1:3 ↔ ISO 4032 M3:34
- Mate:244: Cart_Floor_Bottom:1 ↔ Magnet_Holder:1
- Mate:245: Door:1 ↔ Lever:1
- Mate:246: Door:1 ↔ Lever:2
- Flush:9: Cart_Floor_Bottom:1 ↔ Door_LimitSwitch_Offset:1
- Mate:247: Cart_Floor_Bottom:1 ↔ Door_LimitSwitch_Offset:2
- Mate:248 (12 mm): Door_LimitSwitch_Offset:1 ↔ Door_LimitSwitch_Offset:2
- Flush:10: Door_LimitSwitch_Offset:1 ↔ Door_LimitSwitch_Offset:2
- Mate:249: LimitSwitch_Small:2 ↔ Door_LimitSwitch_Offset:1
- Mate:250: LimitSwitch_Small:1 ↔ Door_LimitSwitch_Offset:2
- Mate:251: LimitSwitch_Small:1 ↔ Door_LimitSwitch_Offset:2
- Mate:252: LimitSwitch_Small:1 ↔ Door_LimitSwitch_Offset:2
- Mate:253: LimitSwitch_Small:2 ↔ Door_LimitSwitch_Offset:1
- Mate:254: LimitSwitch_Small:2 ↔ Door_LimitSwitch_Offset:1
- Mate:255: LimitSwitch_Small:4 ↔ LimitSwitch_Small:2
- Mate:256: LimitSwitch_Small:4 ↔ LimitSwitch_Small:2
- Mate:257: LimitSwitch_Small:4 ↔ LimitSwitch_Small:2
- Mate:258: LimitSwitch_Small:1 ↔ LimitSwitch_Small:3
- Mate:259: LimitSwitch_Small:1 ↔ LimitSwitch_Small:3
- Mate:260: LimitSwitch_Small:1 ↔ LimitSwitch_Small:3
- Mate:261: Cart_Floor:1 ↔ Car_Rear:1
- Mate:262: Car_Left:1 ↔ Car_Rear:1
- Mate:263: Cart_Floor:1 ↔ Car_Left:1
- Mate:264: Car_Left:1 ↔ Cart_Floor_Bottom:1
- Mate:265: Cart_Floor_Bottom:1 ↔ Spindle_Block_ASM_MIR:1
- Mate:266: Cart_Floor_Bottom:1 ↔ Spindle_Block_ASM_MIR:1
- Mate:267: Cart_Floor_Bottom:1 ↔ Bearing_ASM_MIR1:2
- Mate:268: Cart_Floor_Bottom:1 ↔ Bearing_ASM_MIR1:2
- Mate:269: Cart_Floor_Bottom:1 ↔ ISO 1207 M3 x 12:36
- Mate:270: Cart_Floor_Bottom:1 ↔ ISO 1207 M3 x 12:38
- Mate:271: Cart_Floor_Bottom:1 ↔ Bearing_ASM_MIR1:1
- Mate:272: Cart_Floor_Bottom:1 ↔ Bearing_ASM_MIR1:3
- Mate:273: Cart_Floor_Bottom:1 ↔ Bearing_ASM_MIR1:3
- Mate:274: Cart_Floor_Bottom:1 ↔ Bearing_ASM_MIR1:1
- Mate:275: Cart_Floor_Bottom:1 ↔ ISO 1207 M3 x 12:42
- Mate:276: Cart_Floor_Bottom:1 ↔ ISO 1207 M3 x 12:31
- Mate:277: Cart_Floor_Bottom:1 ↔ ISO 4032 M3:33
- Flush:11: ISO 4032 M3:31 ↔ ISO 4032 M3:33
- Flush:12: ISO 4032 M3:33 ↔ ISO 4032 M3:34
- Flush:13: ISO 4032 M3:32 ↔ ISO 4032 M3:34
- Flush:14: ISO 4032 M3:29 ↔ ISO 4032 M3:31
- Flush:15: ISO 4032 M3:30 ↔ ISO 4032 M3:33
- Flush:16: ISO 4032 M3:31 ↔ ISO 4032 M3:33
- Flush:17: ISO 4032 M3:31 ↔ ISO 4032 M3:36
- Flush:18: ISO 4032 M3:35 ↔ ISO 4032 M3:36
- Flush:19: ISO 4032 M3:36 ↔ ISO 4032 M3:50
- Flush:20: ISO 4032 M3:50 ↔ ISO 4032 M3:51
- Flush:21: ISO 4032 M3:35 ↔ ISO 4032 M3:37
- Flush:22: ISO 4032 M3:37 ↔ ISO 4032 M3:47
- Flush:23: ISO 4032 M3:47 ↔ ISO 4032 M3:48
- Flush:24: ISO 4032 M3:39 ↔ ISO 4032 M3:51
- Flush:25: ISO 4032 M3:51 ↔ ISO 4032 M3:52
- Flush:26: ISO 4032 M3:38 ↔ ISO 4032 M3:52
- Flush:27: ISO 4032 M3:39 ↔ ISO 4032 M3:40
- Flush:28: ISO 4032 M3:40 ↔ ISO 4032 M3:49
- Flush:29: ISO 4032 M3:44 ↔ ISO 4032 M3:45
- Flush:30: ISO 4032 M3:42 ↔ ISO 4032 M3:44
- Flush:31: ISO 4032 M3:41 ↔ ISO 4032 M3:42
- Flush:32: ISO 4032 M3:41 ↔ ISO 4032 M3:43
- Flush:33: ISO 4032 M3:43 ↔ ISO 4032 M3:46
- Flush:34: ISO 4032 M3:40 ↔ ISO 4032 M3:44
- Mate:278: Cart_Floor:1 ↔ Magnet_Holder:1
- Mate:279: Cart_Floor_Bottom:1 ↔ Magnet_Holder:1
- Mate:280: Cart_Floor_Bottom:1 ↔ Magnet_Holder:1
- Mate:281: Cart_Floor_Bottom:1 ↔ LimitSwitch_Small:3
- Mate:282: Cart_Floor_Bottom:1 ↔ LimitSwitch_Small:3
- Mate:283: Cart_Floor_Bottom:1 ↔ LimitSwitch_Small:4
- Mate:284: Cart_Floor_Bottom:1 ↔ LimitSwitch_Small:4
- Flush:35: Cart_Floor_Bottom:1 ↔ Door_LimitSwitch_Holder_Side_1:1
- Mate:285: Cart_Floor_Bottom:1 ↔ Door_LimitSwitch_Holder_Side_1:1
- Mate:286: Cart_Floor_Bottom:1 ↔ Door_LimitSwitch_Holder_Side_1:1
- Mate:287: Cart_Floor_Bottom:1 ↔ Door_LimitSwitch_Holder_Side_1:1
- Flush:36: Cart_Floor_Bottom:1 ↔ Door_LimitSwitch_Holder_Side_2:1
- Mate:288: Cart_Floor_Bottom:1 ↔ Door_LimitSwitch_Holder_Side_2:1
- Mate:289: Door_LimitSwitch_Holder_Side_1:1 ↔ Door_LimitSwitch_Holder_Side_2:1
- Flush:37: Door_LimitSwitch_Holder_Side_1:1 ↔ Door_LimitSwitch_Holder_Side_2:1
- Flush:38: Door_LimitSwitch_Holder_Side_1:1 ↔ Door_LimitSwitch_Holder_Plate:1
- Mate:290: LimitSwitch_Small:5 ↔ Door_LimitSwitch_Holder_Plate:1
- Mate:291: LimitSwitch_Small:5 ↔ Door_LimitSwitch_Holder_Plate:1
- Mate:292: LimitSwitch_Small:5 ↔ Door_LimitSwitch_Holder_Plate:1
- Mate:293: Door_LimitSwitch_Holder_Side_2:1 ↔ Door_LimitSwitch_Holder_Plate:1
- Flush:39: Door_LimitSwitch_Holder_Side_1:1 ↔ Door_LimitSwitch_Holder_Plate:1
- Flush:40: Door_LimitSwitch_Holder_Side_2:1 ↔ Door_LimitSwitch_Holder_Plate:1
- Mate:294 (4.6 mm): Lever:3 ↔ LimitSwitch_Small:5
- Mate:295: Door:1 ↔ Lever:5
- Mate:296: Door:1 ↔ Lever:5
- Mate:297: Door:1 ↔ Lever:5
- Mate:298: Lever:4 ↔ Lever:6
- Mate:299: Door_MIR:1 ↔ Lever:6
- Mate:300: Door_MIR:1 ↔ Lever:6
- Mate:301: Lever:3 ↔ LimitSwitch_Small:5
- Symmetry:2: Car_Left:1 ↔ Car_Right:2
- Flush:41: Door_LimitSwitch_Holder_Side_1_MIR:1 ↔ Door_LimitSwitch_Holder_Side_2_MIR:1
- Mate:302: Door_LimitSwitch_Holder_Side_1_MIR:1 ↔ Door_LimitSwitch_Holder_Side_2_MIR:1
- Flush:42: Door_LimitSwitch_Holder_Side_2_MIR:1 ↔ Door_LimitSwitch_Holder_Plate_MIR:1
- Flush:43: Door_LimitSwitch_Holder_Side_1_MIR:1 ↔ Door_LimitSwitch_Holder_Plate_MIR:1
- Mate:303: Door_LimitSwitch_Holder_Side_2_MIR:1 ↔ Door_LimitSwitch_Holder_Plate_MIR:1
- Mate:304: Door_LimitSwitch_Holder_Side_1_MIR:1 ↔ Door_LimitSwitch_Holder_Plate_MIR:1
- Mate:305: Cart_Floor_Bottom:1 ↔ Door_LimitSwitch_Holder_Side_1_MIR:1
- Flush:44: Door_LimitSwitch_Holder_Side_1_MIR:1 ↔ Door_LimitSwitch_Holder_Side_2_MIR:1
- Mate:307: Cart_Floor_Bottom:1 ↔ Door_LimitSwitch_Holder_Side_1_MIR:1
- Mate:308: LimitSwitch_Small:6 ↔ Door_LimitSwitch_Holder_Plate_MIR:1
- Mate:309: LimitSwitch_Small:6 ↔ Door_LimitSwitch_Holder_Plate_MIR:1
- Mate:310: LimitSwitch_Small:6 ↔ Door_LimitSwitch_Holder_Plate_MIR:1
- Mate:311: Lever:2 ↔ LimitSwitch_Small:6
- Mate:312: Door:1 ↔ ISO 1207 M3 x 12:53
- Mate:313: Door:1 ↔ ISO 1207 M3 x 12:53
- Mate:314: Door:1 ↔ ISO 4032 M3:53
- Mate:315: Lever:5 ↔ ISO 4032 M3:53
- Mate:316: Door:1 ↔ ISO 1207 M3 x 12:54
- Mate:317: Door:1 ↔ ISO 1207 M3 x 12:54
- Mate:318: Door:1 ↔ ISO 4032 M3:54
- Mate:319: Lever:2 ↔ ISO 4032 M3:54
- Mate:320: Door_MIR:1 ↔ ISO 1207 M3 x 12:55
- Mate:321: Door_MIR:1 ↔ ISO 1207 M3 x 12:55
- Mate:322: Door_MIR:1 ↔ ISO 4032 M3:55
- Mate:323: Lever:3 ↔ ISO 4032 M3:55
- Mate:324: Door_MIR:1 ↔ ISO 1207 M3 x 12:56
- Mate:325: Door_MIR:1 ↔ ISO 1207 M3 x 12:56
- Mate:326: Door_MIR:1 ↔ ISO 4032 M3:56
- Mate:327: Lever:6 ↔ ISO 4032 M3:56
- Mate:328: LimitSwitch_Small:3 ↔ AS 1427 (8) - Metric M2 x 25:1
- Mate:329: LimitSwitch_Small:3 ↔ AS 1427 (8) - Metric M2 x 25:1
- Mate:330: LimitSwitch_Small:3 ↔ ISO 7089 2:1
- Mate:331: Cart_Floor_Bottom:1 ↔ ISO 7089 2:1
- Insert:5: ISO 7089 2:1 ↔ ISO 4032 M2:1
- Mate:332: LimitSwitch_Small:3 ↔ AS 1427 (8) - Metric M2 x 25:2
- Mate:333: LimitSwitch_Small:3 ↔ AS 1427 (8) - Metric M2 x 25:2
- Mate:334: LimitSwitch_Small:3 ↔ ISO 7089 2:2
- Mate:335: Cart_Floor_Bottom:1 ↔ ISO 7089 2:2
- Insert:6: ISO 7089 2:2 ↔ ISO 4032 M2:2
- Mate:336: LimitSwitch_Small:4 ↔ AS 1427 (8) - Metric M2 x 25:3
- Mate:337: LimitSwitch_Small:4 ↔ AS 1427 (8) - Metric M2 x 25:3
- Mate:338: LimitSwitch_Small:4 ↔ ISO 7089 2:3
- Mate:339: Cart_Floor_Bottom:1 ↔ ISO 7089 2:3
- Insert:7: ISO 7089 2:3 ↔ ISO 4032 M2:3
- Mate:340: LimitSwitch_Small:4 ↔ AS 1427 (8) - Metric M2 x 25:4
- Mate:341: LimitSwitch_Small:4 ↔ AS 1427 (8) - Metric M2 x 25:4
- Mate:342: LimitSwitch_Small:4 ↔ ISO 7089 2:4
- Mate:343: Cart_Floor_Bottom:1 ↔ ISO 7089 2:4
- Insert:8: ISO 7089 2:4 ↔ ISO 4032 M2:4
- Mate:344: LimitSwitch_Small:6 ↔ AS 1427 (8) - Metric M2 x 16:1
- Mate:345: LimitSwitch_Small:6 ↔ AS 1427 (8) - Metric M2 x 16:1
- Mate:346: LimitSwitch_Small:6 ↔ ISO 7089 2:5
- Mate:347: Door_LimitSwitch_Holder_Plate_MIR:1 ↔ ISO 7089 2:5
- Insert:9: ISO 7089 2:5 ↔ ISO 4032 M2:5
- Mate:348: LimitSwitch_Small:6 ↔ AS 1427 (8) - Metric M2 x 16:2
- Mate:349: LimitSwitch_Small:6 ↔ AS 1427 (8) - Metric M2 x 16:2
- Mate:350: LimitSwitch_Small:6 ↔ ISO 7089 2:6
- Mate:351: Door_LimitSwitch_Holder_Plate_MIR:1 ↔ ISO 7089 2:6
- Insert:10: ISO 7089 2:6 ↔ ISO 4032 M2:6
- Mate:352: LimitSwitch_Small:5 ↔ AS 1427 (8) - Metric M2 x 16:3
- Mate:353: LimitSwitch_Small:5 ↔ AS 1427 (8) - Metric M2 x 16:3
- Mate:354: LimitSwitch_Small:5 ↔ ISO 7089 2:7
- Mate:355: Door_LimitSwitch_Holder_Plate:1 ↔ ISO 7089 2:7
- Insert:11: ISO 7089 2:7 ↔ ISO 4032 M2:7
- Mate:356: LimitSwitch_Small:5 ↔ AS 1427 (8) - Metric M2 x 16:4
- Mate:357: LimitSwitch_Small:5 ↔ AS 1427 (8) - Metric M2 x 16:4
- Mate:358: LimitSwitch_Small:5 ↔ ISO 7089 2:8
- Mate:359: Door_LimitSwitch_Holder_Plate:1 ↔ ISO 7089 2:8
- Insert:12: ISO 7089 2:8 ↔ ISO 4032 M2:8
- Mate:360: Cart_Floor_Bottom:1 ↔ ISO 1207 M3 x 12:57
- Mate:361: Cart_Floor_Bottom:1 ↔ ISO 1207 M3 x 12:57
- Mate:362: Cart_Floor_Bottom:1 ↔ ISO 4032 M3:57
- Mate:363: Door_LimitSwitch_Holder_Side_2:1 ↔ ISO 4032 M3:57
- Mate:364: Cart_Floor_Bottom:1 ↔ ISO 1207 M3 x 12:58
- Mate:365: Cart_Floor_Bottom:1 ↔ ISO 1207 M3 x 12:58
- Mate:366: Cart_Floor_Bottom:1 ↔ ISO 4032 M3:58
- Mate:367: Door_LimitSwitch_Holder_Side_1:1 ↔ ISO 4032 M3:58
- Mate:368: Door_LimitSwitch_Holder_Plate:1 ↔ ISO 1207 M3 x 12:59
- Mate:369: Door_LimitSwitch_Holder_Plate:1 ↔ ISO 1207 M3 x 12:59
- Mate:370: Door_LimitSwitch_Holder_Plate:1 ↔ ISO 4032 M3:59
- Mate:371: Door_LimitSwitch_Holder_Side_1:1 ↔ ISO 4032 M3:59
- Mate:372: Door_LimitSwitch_Holder_Plate:1 ↔ ISO 1207 M3 x 12:60
- Mate:373: Door_LimitSwitch_Holder_Plate:1 ↔ ISO 1207 M3 x 12:60
- Mate:374: Door_LimitSwitch_Holder_Plate:1 ↔ ISO 4032 M3:60
- Mate:375: Door_LimitSwitch_Holder_Side_2:1 ↔ ISO 4032 M3:60
- Mate:376: Cart_Floor_Bottom:1 ↔ ISO 1207 M3 x 12:61
- Mate:377: Cart_Floor_Bottom:1 ↔ ISO 1207 M3 x 12:61
- Mate:378: Cart_Floor_Bottom:1 ↔ ISO 4032 M3:61
- Mate:379: Door_LimitSwitch_Holder_Side_2_MIR:1 ↔ ISO 4032 M3:61
- Mate:380: Cart_Floor_Bottom:1 ↔ Door_LimitSwitch_Holder_Side_1_MIR:1
- Mate:381: Cart_Floor_Bottom:1 ↔ ISO 1207 M3 x 12:62
- Mate:382: Cart_Floor_Bottom:1 ↔ ISO 1207 M3 x 12:62
- Mate:383: Cart_Floor_Bottom:1 ↔ ISO 4032 M3:62
- Mate:384: Door_LimitSwitch_Holder_Side_1_MIR:1 ↔ ISO 4032 M3:62
- Mate:385: Door_LimitSwitch_Holder_Plate_MIR:1 ↔ ISO 1207 M3 x 12:63
- Mate:386: Door_LimitSwitch_Holder_Plate_MIR:1 ↔ ISO 1207 M3 x 12:63
- Mate:387: Door_LimitSwitch_Holder_Plate_MIR:1 ↔ ISO 4032 M3:63
- Mate:388: Door_LimitSwitch_Holder_Side_1_MIR:1 ↔ ISO 4032 M3:63
- Mate:389: Door_LimitSwitch_Holder_Plate_MIR:1 ↔ ISO 1207 M3 x 12:64
- Mate:390: Door_LimitSwitch_Holder_Plate_MIR:1 ↔ ISO 1207 M3 x 12:64
- Mate:391: Door_LimitSwitch_Holder_Plate_MIR:1 ↔ ISO 4032 M3:64
- Mate:392: Door_LimitSwitch_Holder_Side_2_MIR:1 ↔ ISO 4032 M3:64
- Mate:393: Cart_Floor:1 ↔ ISO 1207 M3 x 12:65
- Mate:394: Cart_Floor:1 ↔ ISO 1207 M3 x 12:65
- Mate:395: Cart_Floor:1 ↔ ISO 4032 M3:65
- Mate:396: Magnet_Holder:1 ↔ ISO 4032 M3:65
- Angle:1 (0 deg): ISO 4032 M3:62 ↔ ISO 4032 M3:63
- Angle:2 (0 deg): Door_LimitSwitch_Holder_Side_1_MIR:1 ↔ ISO 4032 M3:63
- Angle:3 (0 deg): Door_LimitSwitch_Holder_Side_2_MIR:1 ↔ ISO 4032 M3:64
- Angle:4 (0 deg): ISO 4032 M3:61 ↔ ISO 4032 M3:64
- Angle:5 (0 deg): ISO 4032 M3:53 ↔ ISO 4032 M3:54
- Angle:6 (0 deg): Lever:5 ↔ ISO 4032 M3:53
- Angle:7 (0 deg): ISO 4032 M3:57 ↔ ISO 4032 M3:60
- Angle:8 (0 deg): Door_LimitSwitch_Holder_Side_2:1 ↔ ISO 4032 M3:57
- Angle:9 (0 deg): ISO 4032 M3:58 ↔ ISO 4032 M3:59
- Angle:10 (0 deg): Door_LimitSwitch_Holder_Side_1:1 ↔ ISO 4032 M3:58
- Angle:11 (0 deg): ISO 4032 M3:53 ↔ ISO 4032 M3:54
- Mate:397: Car_Rear:1 ↔ ISO 1207 M3 x 12:66
- Mate:398: Car_Rear:1 ↔ ISO 1207 M3 x 12:66
- Mate:399: Car_Rear:1 ↔ ISO 1207 M3 x 12:67
- Mate:400: Car_Rear:1 ↔ ISO 1207 M3 x 12:67
- Mate:401: Car_Rear:1 ↔ ISO 4032 M3:66
- Mate:402: Car_Right:2 ↔ ISO 4032 M3:66
- Mate:403: Car_Rear:1 ↔ ISO 4032 M3:67
- Mate:404: Car_Right:2 ↔ ISO 4032 M3:67
- Mate:405: Cart_Floor:1 ↔ ISO 1207 M3 x 12:68
- Mate:406: Cart_Floor:1 ↔ ISO 1207 M3 x 12:68
- Mate:407: Cart_Floor:1 ↔ ISO 1207 M3 x 12:69
- Mate:408: Cart_Floor:1 ↔ ISO 1207 M3 x 12:69
- Mate:409: Cart_Floor:1 ↔ ISO 1207 M3 x 12:70
- Mate:410: Cart_Floor:1 ↔ ISO 1207 M3 x 12:70
- Mate:411: Cart_Floor:1 ↔ ISO 4032 M3:68
- Mate:412: Car_Left:1 ↔ ISO 4032 M3:68
- Mate:413: Cart_Floor:1 ↔ ISO 4032 M3:69
- Mate:414: Car_Left:1 ↔ ISO 4032 M3:69
- Mate:415: Cart_Floor:1 ↔ ISO 4032 M3:70
- Mate:416: Car_Left:1 ↔ ISO 4032 M3:70
- Mate:417: Cart_Floor_Bottom:1 ↔ ISO 1207 M3 x 12:71
- Mate:418: Cart_Floor_Bottom:1 ↔ ISO 1207 M3 x 12:71
- Mate:419: Cart_Floor_Bottom:1 ↔ ISO 1207 M3 x 12:72
- Mate:420: Cart_Floor_Bottom:1 ↔ ISO 1207 M3 x 12:72
- Mate:421: Cart_Floor_Bottom:1 ↔ ISO 1207 M3 x 12:73
- Mate:422: Cart_Floor_Bottom:1 ↔ ISO 1207 M3 x 12:73
- Mate:423: Cart_Floor_Bottom:1 ↔ ISO 4032 M3:71
- Mate:424: Car_Rear:1 ↔ ISO 4032 M3:71
- Mate:425: Cart_Floor_Bottom:1 ↔ ISO 4032 M3:72
- Mate:426: Car_Rear:1 ↔ ISO 4032 M3:72
- Mate:427: Cart_Floor_Bottom:1 ↔ ISO 4032 M3:73
- Mate:428: Car_Rear:1 ↔ ISO 4032 M3:73
- Angle:12 (0 deg): Car_Right:2 ↔ ISO 4032 M3:73
- Angle:13 (0 deg): Car_Left:1 ↔ ISO 4032 M3:72
- Angle:14 (0 deg): Car_Right:2 ↔ ISO 4032 M3:70
- Angle:15 (0 deg): Car_Left:1 ↔ ISO 4032 M3:68
- Angle:16 (0 deg): Car_Right:2 ↔ ISO 4032 M3:66
- Angle:17 (0 deg): Car_Rear:1 ↔ ISO 4032 M3:69
- Angle:18 (0 deg): Car_Rear:1 ↔ ISO 4032 M3:71
- Angle:19 (0 deg): Magnet_Holder:1 ↔ ISO 4032 M3:65
- Angle:20 (90 deg): Receptacle:1 ↔ ISO 1207 M3 x 12:6
- Angle:21 (90 deg): Receptacle_MIR:1 ↔ ISO 1207 M3 x 12:19
- Angle:22 (0 deg): ISO 1207 M3 x 12:18 ↔ ISO 1207 M3 x 12:19
- Angle:23 (0 deg): Receptacle_MIR:1 ↔ ISO 4032 M3:32
- Angle:24 (0 deg): ISO 4032 M3:30 ↔ ISO 4032 M3:32
- Angle:25 (0 deg): ISO 4032 M3:32 ↔ ISO 4032 M3:34
- Angle:26 (0 deg): ISO 1207 M3 x 12:69 ↔ ISO 1207 M3 x 12:6
- Mate:429: Cart_Floor:1 ↔ ISO 1207 M3 x 8:3
- Mate:430: Cart_Floor:1 ↔ ISO 1207 M3 x 8:3
- Mate:431: Cart_Floor:1 ↔ ISO 1207 M3 x 8:4
- Mate:432: Cart_Floor:1 ↔ ISO 1207 M3 x 8:4
- Mate:433: Servo_Motor:1 ↔ ISO 1207 M3 x 8:1
- Mate:434: Servo_Motor:1 ↔ ISO 1207 M3 x 8:2
- Mate:435: Servo_Motor:1 ↔ ISO 1207 M3 x 8:1
- Mate:436: Servo_Motor:2 ↔ ISO 1207 M3 x 8:4
- Mate:437: Servo_Motor:2 ↔ ISO 1207 M3 x 8:3
- Mate:438: Receptacle_MIR:1 ↔ ISO 1207 M3 x 12:74
- Mate:439: Receptacle_MIR:1 ↔ ISO 1207 M3 x 12:74
- Mate:440: Receptacle_MIR:1 ↔ ISO 1207 M3 x 12:75
- Mate:441: Receptacle_MIR:1 ↔ ISO 1207 M3 x 12:75
- Mate:442: Receptacle_MIR:1 ↔ ISO 1207 M3 x 12:76
- Mate:443: Receptacle_MIR:1 ↔ ISO 1207 M3 x 12:76
- Mate:444: Receptacle_MIR:1 ↔ ISO 7089 3:5
- Mate:445: Cart_Floor:1 ↔ ISO 7089 3:5
- Mate:446: Receptacle_MIR:1 ↔ ISO 7089 3:6
- Mate:447: Cart_Floor:1 ↔ ISO 7089 3:6
- Mate:448: Receptacle_MIR:1 ↔ ISO 7089 3:7
- Mate:449: Cart_Floor:1 ↔ ISO 7089 3:7
- Insert:13: ISO 7089 3:5 ↔ ISO 4032 M3:74
- Insert:14: ISO 7089 3:6 ↔ ISO 4032 M3:75
- Insert:15: ISO 7089 3:7 ↔ ISO 4032 M3:76
- Mate:450: Receptacle_MIR:1 ↔ Cart_Floor:1
- Mate:451: Receptacle_MIR:1 ↔ Cart_Floor:1
- Mate:452: Receptacle_MIR:1 ↔ ISO 1207 M3 x 12:77
- Mate:453: Receptacle_MIR:1 ↔ ISO 1207 M3 x 12:77
- Mate:454: Receptacle_MIR:1 ↔ ISO 7089 3:8
- Mate:455: Cart_Floor:1 ↔ ISO 7089 3:8
- Insert:16: ISO 7089 3:8 ↔ ISO 4032 M3:77
